# Autodesk Inventor assembly: Calosc(podstawa do poprawy)
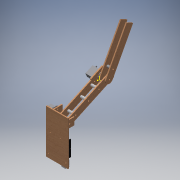
[picture p0: Inventor's stored thumbnail of the model, 180x180]
Saved by Autodesk Inventor 2017 (Build 210142000, 142)
## iProperties
Part Number: Calosc(podstawa do poprawy)
Material: Ogólny
Document SubType Name: Assembly
Designer: Damian
Author: Damian
## Documents named in this file (4)
- C:\Users\Damian\Documents\Inventor\Nowe\2.0\Calosc(podstawa do poprawy).iam
- C:\Users\Damian\Documents\Inventor\Nowe\2.0\Segment_1.iam
- C:\Users\Damian\Documents\Inventor\Nowe\2.0\Segment_2.iam
- C:\Users\Damian\Documents\Inventor\Nowe\2.0\Podstawa-ok.iam
## Components (3 placed, 3 different names)
1. Segment_1:1 [sub-assembly] — Wstaw:2, Wstaw:3
2. Segment_2:1 [sub-assembly] — Wstaw:2
3. Podstawa-ok:1 [sub-assembly] — Wstaw:3
## Relationships (2: Insert 2)
- Wstaw:2 [Insert]: Segment_1:1 ↔ Segment_2:1
- Wstaw:3 [Insert]: Segment_1:1 ↔ Podstawa-ok:1
